# Autodesk Inventor assembly: motor unit 2820
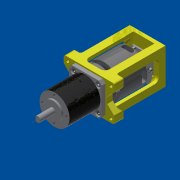
[picture p0: Inventor's stored thumbnail of the model, 180x180]
Saved by Autodesk Inventor 2018 (Build 220112000, 112)
## iProperties
Created: 2020-06-06
Part Number: motor unit 2820
Document SubType Name: Assembly
Designer: Bunny320
Author: Bunny320
## Documents named in this file (13)
- C:\Users\Bunny320\Desktop\sechs\4-CAD\motor unit 2820 (J1).iam
- C:\Users\Bunny320\Desktop\sechs\4-CAD\standardParts\AS 2820 kv880\AS 2820 kv880.ipt
- C:\Users\Bunny320\Desktop\sechs\4-CAD\912-35-reducer.ipt
- C:\Users\Bunny320\Desktop\sechs\4-CAD\922-2820 magnet hold.ipt
- C:\Users\Bunny320\Desktop\sechs\4-CAD\923-2820 back.ipt
- C:\Users\Bunny320\Desktop\sechs\4-CAD\magnet-6x2.5.ipt
- C:\Users\Bunny320\Desktop\sechs\4-CAD\AS5047.ipt
- C:\Users\Bunny320\Documents\Inventor\Content Center Files\R2018\en-US\ISO 4762(1)\DIN EN ISO 4762 - M3 x 8.ipt
- C:\Users\Bunny320\Documents\Inventor\Content Center Files\R2018\en-US\ISO 4762(1)\DIN EN ISO 4762 - M3 x 16.ipt
- C:\Users\Bunny320\Documents\Inventor\Content Center Files\R2018\en-US\ISO 4762(1)\DIN EN ISO 4762 - M2 x 6.ipt
- C:\Users\Bunny320\Documents\Inventor\Content Center Files\R2018\en-US\DIN EN ISO 4032\DIN EN ISO 4032 - M2.ipt
- C:\Users\Bunny320\Documents\Inventor\Content Center Files\R2018\en-US\ISO 4762(1)\DIN EN ISO 4762 - M2.5 x 8.ipt
- C:\Users\Bunny320\Desktop\sechs\4-CAD\921-2820 house (J1).ipt
## Components (26 placed, 12 different names)
1. 921-2820 house (J1):1 — Flush:1, Flush:2, Flush:3, Mate:1, Mate:2, Mate:3, Mate:4, Mate:5, Mate:6, Flush:4, Flush:5, Mate:12, Insert:2
2. AS 2820 kv880:1 — Mate:4, Mate:5, Mate:6, Mate:7, Mate:8, Mate:9
3. 912-35-reducer:1 — Mate:1, Mate:2, Mate:3
4. 922-2820 magnet hold:1 — Mate:7, Mate:8, Mate:9, Mate:13, Mate:14, Insert:7
5. 923-2820 back:1 — Flush:4, Flush:5, Mate:12, Mate:15, Mate:16, Mate:17, Mate:18, Mate:19, Insert:3, Insert:4, Insert:5, Mate:20, Mate:22, Mate:24, Mate:26, Mate:29, Mate:31, Mate:33, Insert:6
6. magnet-6x2.5:1 — Mate:13, Mate:14
7. AS5047:1 — Mate:15, Mate:16, Mate:17, Mate:21, Mate:23, Mate:25, Mate:27
8. DIN EN ISO 4762 M3 x 16:1 — Mate:18, Mate:19
9. DIN EN ISO 4762 M3 x 16:2 — Insert:3
10. DIN EN ISO 4762 M3 x 16:3 — Insert:4
11. DIN EN ISO 4762 M3 x 16:4 — Insert:5
12. DIN EN ISO 4762 M2 x 6:1 — Mate:20, Mate:21
13. DIN EN ISO 4762 M2 x 6:2 — Mate:22, Mate:23, Mate:28
14. DIN EN ISO 4762 M2 x 6:3 — Mate:24, Mate:25, Mate:30
15. DIN EN ISO 4762 M2 x 6:4 — Mate:26, Mate:27, Mate:32
16. DIN EN ISO 4032 M2:1 — Mate:28, Mate:29
17. DIN EN ISO 4032 M2:2 — Mate:30, Mate:31
18. DIN EN ISO 4032 M2:3 — Mate:32, Mate:33
19. DIN EN ISO 4032 M2:4 — Insert:6
20. DIN EN ISO 4762 M3 x 8:2 — Insert:2
21. DIN EN ISO 4762 M3 x 8:3
22. DIN EN ISO 4762 M3 x 8:4
23. DIN EN ISO 4762 M3 x 8:5
24. DIN EN ISO 4762 M2.5 x 8:1 — Insert:7
25. DIN EN ISO 4762 M2.5 x 8:2
26. DIN EN ISO 4762 M2.5 x 8:3
## Component patterns: (4 elements, first: DIN EN ISO 4762 M3 x 8:2), (3 elements, first: DIN EN ISO 4762 M2.5 x 8:1)
## Relationships (42: Mate 31, Insert 6, Flush 5)
- Flush:1: 921-2820 house (J1):1
- Flush:2: 921-2820 house (J1):1
- Flush:3: 921-2820 house (J1):1
- Mate:1: 921-2820 house (J1):1 ↔ 912-35-reducer:1
- Mate:2: 921-2820 house (J1):1 ↔ 912-35-reducer:1
- Mate:3: 921-2820 house (J1):1 ↔ 912-35-reducer:1
- Mate:4: 921-2820 house (J1):1 ↔ AS 2820 kv880:1
- Mate:5: 921-2820 house (J1):1 ↔ AS 2820 kv880:1
- Mate:6: 921-2820 house (J1):1 ↔ AS 2820 kv880:1
- Mate:7: AS 2820 kv880:1 ↔ 922-2820 magnet hold:1
- Mate:8: AS 2820 kv880:1 ↔ 922-2820 magnet hold:1
- Mate:9: AS 2820 kv880:1 ↔ 922-2820 magnet hold:1
- Flush:4: 921-2820 house (J1):1 ↔ 923-2820 back:1
- Flush:5: 921-2820 house (J1):1 ↔ 923-2820 back:1
- Mate:12: 921-2820 house (J1):1 ↔ 923-2820 back:1
- Mate:13: 922-2820 magnet hold:1 ↔ magnet-6x2.5:1
- Mate:14: 922-2820 magnet hold:1 ↔ magnet-6x2.5:1
- Mate:15: 923-2820 back:1 ↔ AS5047:1
- Mate:16: 923-2820 back:1 ↔ AS5047:1
- Mate:17: 923-2820 back:1 ↔ AS5047:1
- Insert:2: 921-2820 house (J1):1 ↔ DIN EN ISO 4762 M3 x 8:2
- Mate:18: 923-2820 back:1 ↔ DIN EN ISO 4762 M3 x 16:1
- Mate:19: 923-2820 back:1 ↔ DIN EN ISO 4762 M3 x 16:1
- Insert:3: 923-2820 back:1 ↔ DIN EN ISO 4762 M3 x 16:2
- Insert:4: 923-2820 back:1 ↔ DIN EN ISO 4762 M3 x 16:3
- Insert:5: 923-2820 back:1 ↔ DIN EN ISO 4762 M3 x 16:4
- Mate:20: 923-2820 back:1 ↔ DIN EN ISO 4762 M2 x 6:1
- Mate:21: AS5047:1 ↔ DIN EN ISO 4762 M2 x 6:1
- Mate:22: 923-2820 back:1 ↔ DIN EN ISO 4762 M2 x 6:2
- Mate:23: AS5047:1 ↔ DIN EN ISO 4762 M2 x 6:2
- Mate:24: 923-2820 back:1 ↔ DIN EN ISO 4762 M2 x 6:3
- Mate:25: AS5047:1 ↔ DIN EN ISO 4762 M2 x 6:3
- Mate:26: 923-2820 back:1 ↔ DIN EN ISO 4762 M2 x 6:4
- Mate:27: AS5047:1 ↔ DIN EN ISO 4762 M2 x 6:4
- Mate:28: DIN EN ISO 4762 M2 x 6:2 ↔ DIN EN ISO 4032 M2:1
- Mate:29: 923-2820 back:1 ↔ DIN EN ISO 4032 M2:1
- Mate:30: DIN EN ISO 4762 M2 x 6:3 ↔ DIN EN ISO 4032 M2:2
- Mate:31: 923-2820 back:1 ↔ DIN EN ISO 4032 M2:2
- Mate:32: DIN EN ISO 4762 M2 x 6:4 ↔ DIN EN ISO 4032 M2:3
- Mate:33: 923-2820 back:1 ↔ DIN EN ISO 4032 M2:3
- Insert:6: 923-2820 back:1 ↔ DIN EN ISO 4032 M2:4
- Insert:7: 922-2820 magnet hold:1 ↔ DIN EN ISO 4762 M2.5 x 8:1
